# Autodesk Inventor assembly: link0
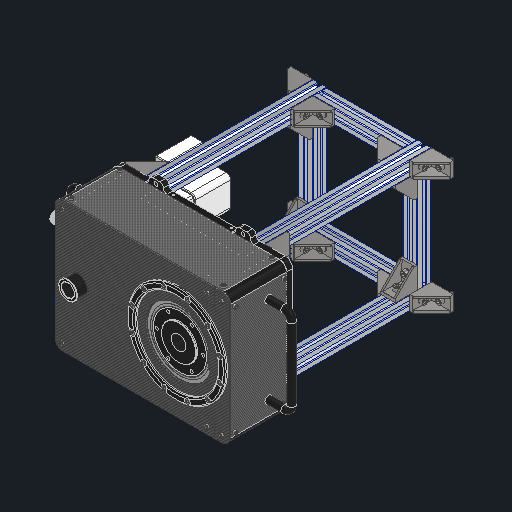
[picture p0: Inventor's stored thumbnail of the model, 512x512]
Saved by Autodesk Inventor 2022 (Build 260153000, 153)
## iProperties
Created: 2021-10-20
Part Number: link0
Document SubType Name: Assembly
Designer: Yuta Kage
Author: Yuta Kage
## Documents named in this file (2)
- C:\Users\yuta0\Documents\GitHub\catchrobo_hardware\mesh\scara\link0.iam
- C:\Users\yuta0\Documents\GitHub\catchrobo_hardware\assy-scara\s-assy-link0.iam
## Components (1 placed, 1 different names)
1. s-assy-link0:2 [sub-assembly] — メイト:1, メイト:2, フラッシュ:1
## Relationships (3: Mate 2, Flush 1)
- メイト:1 [Mate]: s-assy-link0:2
- メイト:2 [Mate]: s-assy-link0:2
- フラッシュ:1 [Flush]: s-assy-link0:2
